# Autodesk Inventor assembly: steering_kingpin_right_assy
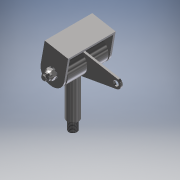
[picture p0: Inventor's stored thumbnail of the model, 180x180]
Saved by Autodesk Inventor 2019 (Build 230136000, 136)
## iProperties
Created: 2019-04-24
Part Number: steering_kingpin_right_assy
Document SubType Name: Assembly
Designer: callum.snowden
Author: callum.snowden
## Documents named in this file (9)
- C:\Users\callum.snowden\Documents\GitHub\clasohlsonkart\mechanical\frame\steering_kingpin_right_assy.iam
- C:\Users\callum.snowden\Documents\GitHub\clasohlsonkart\mechanical\frame\steering_kingpin_right.ipt
- C:\Users\callum.snowden\Documents\GitHub\clasohlsonkart\mechanical\frame\steering_kingpin_bearing_spacer.ipt
- C:\Users\callum.snowden\Documents\Inventor\Content Center Files\R2019\en-US\SKF 2Z - with two shields\SKF 2Z6200-2Z.ipt
- C:\Users\callum.snowden\Documents\Inventor\Content Center Files\R2019\en-US\ANSI B18.16.3M(2)\ANSI B18.16.3M - Property Class 5 and 10 - Metric M8 x 1.25 Top Insert Type.ipt
- C:\Users\callum.snowden\Documents\Inventor\Content Center Files\R2019\en-US\IFI 532(1)\IFI 532 - 8(1) A.ipt
- C:\Users\callum.snowden\Documents\Inventor\Content Center Files\R2019\en-US\BS 4168(7)\BS 4168 - 10 x 70.ipt
- C:\Users\callum.snowden\Documents\GitHub\clasohlsonkart\mechanical\frame\steering_kingpin_bracket.ipt
- C:\Users\callum.snowden\Documents\Inventor\Content Center Files\R2019\en-US\BS 4320(2)\BS 4320 - M10 (Form A).ipt
## Components (10 placed, 8 different names)
1. steering_kingpin_right:1 — Rigid:1, Rigid:3
2. steering_kingpin_bearing_spacer:1 — Rigid:2
3. SKF 2Z- with two shields SKF 2Z6200-2Z:1 — Rigid:1, Rigid:2, Rotational:2
4. SKF 2Z- with two shields SKF 2Z6200-2Z:2 — Rigid:3, Rotational:1
5. Prevailing Torque Type Hex Nut - Steel Metric Property Class 5 and 10 - Metric M8 x 1.25 Top Insert Type:1 — Rotational:6
6. External Tooth Lock Washer - Type A (Metric) (IFI) 8:1 — Rotational:5, Rotational:6
7. BS 4168 : Part 7 Hexagon socket screws and wrench keys, metric series- Specification for hexagon socket shoulder screws - Metric 10 x 70:1 — Rotational:4, Rotational:5
8. steering_kingpin_bracket:1 — Rotational:3, Rotational:4
9. BS 4320 Form AB M10 (Form A):1 — Rotational:2
10. BS 4320 Form AB M10 (Form A):2 — Rotational:1, Rotational:3
## Relationships (9: RevoluteJoint 6, WeldJoint 3)
- Rigid:1 [WeldJoint]: steering_kingpin_right:1 ↔ SKF 2Z- with two shields SKF 2Z6200-2Z:1
- Rigid:2 [WeldJoint]: steering_kingpin_bearing_spacer:1 ↔ SKF 2Z- with two shields SKF 2Z6200-2Z:1
- Rigid:3 [WeldJoint]: steering_kingpin_right:1 ↔ SKF 2Z- with two shields SKF 2Z6200-2Z:2
- Rotational:1 [RevoluteJoint]: SKF 2Z- with two shields SKF 2Z6200-2Z:2 ↔ BS 4320 Form AB M10 (Form A):2
- Rotational:2 [RevoluteJoint]: SKF 2Z- with two shields SKF 2Z6200-2Z:1 ↔ BS 4320 Form AB M10 (Form A):1
- Rotational:3 [RevoluteJoint]: steering_kingpin_bracket:1 ↔ BS 4320 Form AB M10 (Form A):2
- Rotational:4 [RevoluteJoint]: BS 4168 : Part 7 Hexagon socket screws and wrench keys, metric series- Specification for hexagon socket shoulder screws - Metric 10 x 70:1 ↔ steering_kingpin_bracket:1
- Rotational:5 [RevoluteJoint]: External Tooth Lock Washer - Type A (Metric) (IFI) 8:1 ↔ BS 4168 : Part 7 Hexagon socket screws and wrench keys, metric series- Specification for hexagon socket shoulder screws - Metric 10 x 70:1
- Rotational:6 [RevoluteJoint]: Prevailing Torque Type Hex Nut - Steel Metric Property Class 5 and 10 - Metric M8 x 1.25 Top Insert Type:1 ↔ External Tooth Lock Washer - Type A (Metric) (IFI) 8:1
